# Autodesk Inventor assembly: AirPressureValve
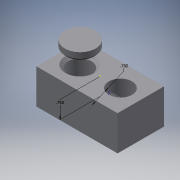
[picture p0: Inventor's stored thumbnail of the model, 180x180]
Saved by Autodesk Inventor 2018 (Build 220112000, 112)
## iProperties
Created: 2020-03-27
Part Number: AirPressureValve
Document SubType Name: Assembly
Designer: emile
Author: emile
## Documents named in this file (3)
- C:\Users\emile\OneDrive\Documents\Inventor\Respirator\Peep\AirPressureValve.iam
- C:\Users\emile\OneDrive\Documents\Inventor\Respirator\Peep\AirPressureAndValve.ipt
- C:\Users\emile\OneDrive\Documents\Inventor\Respirator\Peep\Diaphragm.iam
## Components (2 placed, 2 different names)
1. AirPressureAndValve:1 — Flush:1, Flush:2, Flush:3, Mate:1
2. Diaphragm:1 [sub-assembly] — Mate:1
## Relationships (4: Flush 3, Mate 1)
- Flush:1: AirPressureAndValve:1
- Flush:2: AirPressureAndValve:1
- Flush:3: AirPressureAndValve:1
- Mate:1: AirPressureAndValve:1 ↔ Diaphragm:1
